# Autodesk Inventor assembly: case
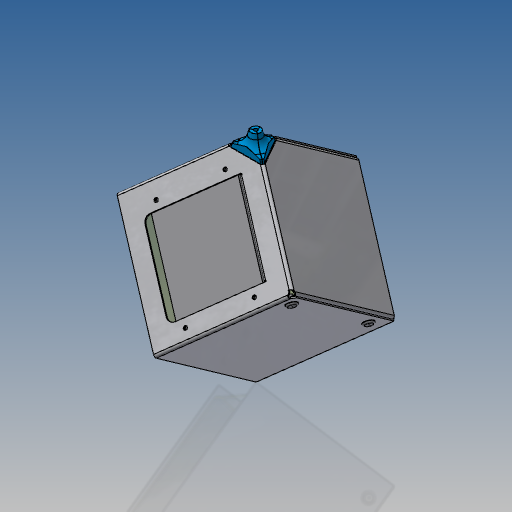
[picture p0: Inventor's stored thumbnail of the model, 512x512]
Saved by Autodesk Inventor 2017 (Build 210142000, 142)
## iProperties
Created: 2017-07-26
Part Number: case
Document SubType Name: Assembly
Designer: leo
Author: leo
## Documents named in this file (7)
- C:\Users\Leo\Dropbox\multiactuador\case.iam
- C:\Users\Leo\Dropbox\multiactuador\case\top.ipt
- C:\Users\Leo\Dropbox\multiactuador\case\traba cable.ipt
- C:\Users\Leo\Dropbox\multiactuador\case\remache.ipt
- C:\Users\Leo\Dropbox\multiactuador\case\base teclado.ipt
- C:\Users\Leo\Dropbox\multiactuador\case\Design Accelerator\Bolted Connection1.iam
- C:\Users\Leo\Dropbox\multiactuador\case\tapa.ipt
## Components (11 placed, 6 different names)
1. top:1 — Angle:1, Angle:2, Mate:1, Mate:2, Insert:1, Insert:2, Insert:3, Insert:4, Flush:2, Mate:3, Flush:3, Mate:4, Mate:5, Flush:4
2. remache:1 — Insert:3
3. remache:2 — Insert:4
4. remache:3 — Insert:1
5. remache:4 — Insert:2
6. base teclado:1 — Flush:2, Mate:3, Flush:3
7. Bolted Connection:1 [sub-assembly] — Mate:4, Mate:5
8. tapa:1 — Flush:4
9. traba cable:1 — Flush:1
10. traba cable:2
11. traba cable:3
## Component patterns: (3 elements, first: traba cable:1)
## Relationships (15: Mate 5, Flush 4, Insert 4, Angle 2)
- Angle:1 (54.74 deg): top:1
- Angle:2 (54.74 deg): top:1
- Mate:1: top:1
- Mate:2: top:1
- Flush:1: traba cable:1
- Insert:1: top:1 ↔ remache:3
- Insert:2: top:1 ↔ remache:4
- Insert:3: top:1 ↔ remache:1
- Insert:4: top:1 ↔ remache:2
- Flush:2 (1 mm): top:1 ↔ base teclado:1
- Mate:3: top:1 ↔ base teclado:1
- Flush:3: top:1 ↔ base teclado:1
- Mate:4: top:1 ↔ Bolted Connection:1
- Mate:5: top:1 ↔ Bolted Connection:1
- Flush:4: top:1 ↔ tapa:1
